# Autodesk Inventor assembly: V1Towers
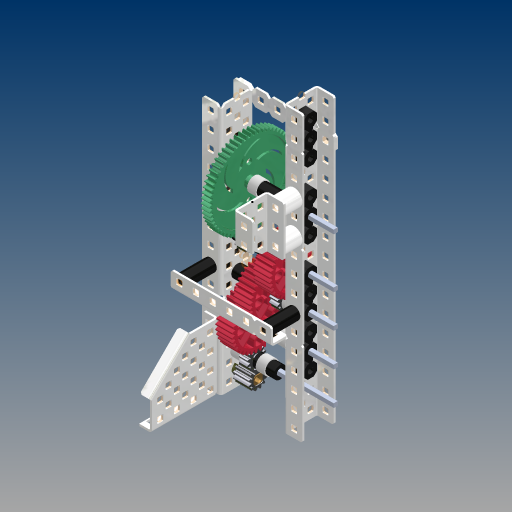
[picture p0: Inventor's stored thumbnail of the model, 512x512]
Saved by Autodesk Inventor 2023 (Build 270158000, 158)
## iProperties
Created: 2023-07-20
Part Number: V1Towers
Document SubType Name: Assembly
Designer: eddie
Author: eddie
## Documents named in this file (26)
- C:\Users\eddie\Documents\81208X-Over-Under-CAD\V1\V1Tower_Right.iam
- C:\Users\eddie\Documents\81208X-Over-Under-CAD\VEX-CAD-Inventor-1.4.0\Motion\Spacers\Spacer Nylon .375 OD\NSpacer .375 OD x .375.ipt
- C:\Users\eddie\Documents\81208X-Over-Under-CAD\VEX-CAD-Inventor-1.4.0\Motion\Spacers\Spacer Nylon .375 OD.ipt
- C:\Users\eddie\Documents\81208X-Over-Under-CAD\VEX-CAD-Inventor-1.4.0\Motion\Spacers\Spacer Nylon .375 OD\NSpacer .375 OD x .500.ipt
- C:\Users\eddie\Documents\81208X-Over-Under-CAD\VEX-CAD-Inventor-1.4.0\Motion\Spacers\Spacer Nylon .500 OD\NSpacer White .500 OD x .500.ipt
- C:\Users\eddie\Documents\81208X-Over-Under-CAD\VEX-CAD-Inventor-1.4.0\Motion\Spacers\Spacer Nylon .500 OD.ipt
- C:\Users\eddie\Documents\81208X-Over-Under-CAD\VEX-CAD-Inventor-1.4.0\Motion\Shaft LS\Shaft LS\Shaft LS 3.0.ipt
- C:\Users\eddie\Documents\81208X-Over-Under-CAD\VEX-CAD-Inventor-1.4.0\Motion\Shaft LS\Shaft LS.ipt
- C:\Users\eddie\Documents\81208X-Over-Under-CAD\VEX-CAD-Inventor-1.4.0\Motion\Spacers\Spacer Nylon .375 OD\NSpacer .375 OD x .125.ipt
- C:\Users\eddie\Documents\81208X-Over-Under-CAD\VEX-CAD-Inventor-1.4.0\Motion\Spacers\Spacer Nylon .375 OD\NSpacer .375 OD x .250.ipt
- C:\Users\eddie\Documents\81208X-Over-Under-CAD\VEX-CAD-Inventor-1.4.0\Motion\Spacers\Washer Steel\SWasher .375 OD x .031250.ipt
- C:\Users\eddie\Documents\81208X-Over-Under-CAD\VEX-CAD-Inventor-1.4.0\Motion\Spacers\Washer Steel.ipt
- C:\Users\eddie\Documents\81208X-Over-Under-CAD\Custom-parts\Angle Corner Gusset.ipt
- C:\Users\eddie\Documents\81208X-Over-Under-CAD\VEX-CAD-Inventor-1.4.0\Structure\C Channel\Aluminum 1x2x1\Alu C 1x2x1x15_MIR.ipt
- C:\Users\eddie\Documents\81208X-Over-Under-CAD\VEX-CAD-Inventor-1.4.0\Structure\C Channel\Aluminum 1x2x1\Alu C 1x2x1x17_MIR.ipt
- C:\Users\eddie\Documents\81208X-Over-Under-CAD\VEX-CAD-Inventor-1.4.0\Structure\Plate\Aluminum\Alu Plate 1x6_MIR.ipt
- C:\Users\eddie\Documents\81208X-Over-Under-CAD\VEX-CAD-Inventor-1.4.0\Structure\Angle\Aluminum\1x1\Alu Angle 1x1x6_MIR.ipt
- C:\Users\eddie\Documents\81208X-Over-Under-CAD\Custom-parts\3x2 channel triangular slice_MIR.ipt
- C:\Users\eddie\Documents\81208X-Over-Under-CAD\VEX-CAD-Inventor-1.4.0\Motion\Shaft LS\Bearing Flat_MIR1.ipt
- C:\Users\eddie\Documents\81208X-Over-Under-CAD\VEX-CAD-Inventor-1.4.0\Structure\Hardware\Nut Alu_MIR.ipt
- C:\Users\eddie\Documents\81208X-Over-Under-CAD\VEX-CAD-Inventor-1.4.0\Motion\Gears\HS Gear\HS 12T Gear, Circle_MIR.iam
- C:\Users\eddie\Documents\81208X-Over-Under-CAD\Custom-parts\Shaft Collar_MIR.ipt
- C:\Users\eddie\Documents\81208X-Over-Under-CAD\VEX-CAD-Inventor-1.4.0\Motion\Gears\LS 12T Gear Steel_MIR.ipt
- C:\Users\eddie\Documents\81208X-Over-Under-CAD\VEX-CAD-Inventor-1.4.0\Motion\Gears\HS Gear\HS 36T Gear, Square_MIR.iam
- C:\Users\eddie\Documents\81208X-Over-Under-CAD\VEX-CAD-Inventor-1.4.0\Motion\Gears\LS 60T Gear_MIR.ipt
- C:\Users\eddie\Documents\81208X-Over-Under-CAD\Custom-parts\Angle Corner Gusset_MIR.ipt
## Components (61 placed, 21 different names)
1. Angle Corner Gusset:1
2. Alu C 1x2x1x15_MIR:1 — Insert:61, Insert:62, Insert:70, Insert:71, Insert:72, Insert:73, Insert:78, Insert:85, Insert:91, Insert:98, Insert:105, Insert:112, Insert:118
3. Alu C 1x2x1x17_MIR:1 — Insert:60, Insert:64, Insert:67, Insert:68, Insert:74, Insert:75, Insert:76, Insert:77, Insert:90
4. Alu Plate 1x6_MIR:1 — Insert:60, Insert:61
5. NSpacer .375 OD x .375:23 — Insert:62, Insert:63
6. NSpacer .375 OD x .500:24 — Insert:63, Insert:66
7. NSpacer .375 OD x .375:25 — Insert:64, Insert:65
8. NSpacer .375 OD x .500:26 — Insert:65
9. Alu Angle 1x1x6_MIR:1 — Insert:66
10. NSpacer White .500 OD x .500:3 — Insert:67, Insert:69
11. NSpacer White .500 OD x .500:4 — Insert:68
12. 3x2 channel triangular slice_MIR:1 — Insert:69
13. Bearing Flat_MIR1:1 — Insert:70, Insert:82, Insert:83
14. Bearing Flat_MIR1:2 — Insert:71, Insert:81
15. Bearing Flat_MIR1:3 — Insert:72, Insert:84
16. Bearing Flat_MIR1:4 — Insert:73, Insert:80
17. Bearing Flat_MIR1:5 — Insert:74
18. Bearing Flat_MIR1:6 — Insert:75
19. Bearing Flat_MIR1:7 — Insert:76
20. Bearing Flat_MIR1:8 — Insert:77
21. Nut Alu_MIR:1 — Insert:78, Insert:79
22. HS 12T Gear, Circle_MIR:1 [sub-assembly] — Insert:79
23. Shaft LS 3.0:6 — Insert:80
24. Shaft LS 3.0:7 — Insert:81
25. Shaft LS 3.0:8 — Insert:82
26. Shaft LS 3.0:9 — Insert:83
27. Shaft LS 3.0:10 — Insert:84
28. Shaft Collar_MIR:1 — Insert:85, Insert:86
29. LS 12T Gear Steel_MIR:1 — Insert:86, Insert:87
30. NSpacer .375 OD x .125:27 — Insert:87, Insert:88
31. Shaft Collar_MIR:2 — Insert:88, Insert:89
32. NSpacer .375 OD x .250:28 — Insert:89
33. Bearing Flat_MIR1:9 — Insert:90
34. NSpacer .375 OD x .125:29 — Insert:91, Insert:92
35. HS 36T Gear, Square_MIR:1 [sub-assembly] — Insert:92, Insert:93
36. LS 12T Gear Steel_MIR:2 — Insert:93, Insert:94
37. NSpacer .375 OD x .375:30 — Insert:94, Insert:95
38. Shaft Collar_MIR:3 — Insert:95, Insert:96
39. NSpacer .375 OD x .125:31 — Insert:96, Insert:97
40. NSpacer .375 OD x .125:32 — Insert:97
41. NSpacer .375 OD x .500:33 — Insert:98, Insert:99
42. SWasher .375 OD x .031250:2 — Insert:99, Insert:100
43. NSpacer .375 OD x .125:34 — Insert:100, Insert:101
44. HS 36T Gear, Square_MIR:2 [sub-assembly] — Insert:101, Insert:102
45. LS 12T Gear Steel_MIR:3 — Insert:102, Insert:103
46. Shaft Collar_MIR:4 — Insert:103, Insert:104
47. NSpacer .375 OD x .125:35 — Insert:104
48. NSpacer .375 OD x .125:36 — Insert:105, Insert:106
49. LS 60T Gear_MIR:1 — Insert:106, Insert:107
50. Shaft Collar_MIR:5 — Insert:107, Insert:108
51. NSpacer .375 OD x .375:37 — Insert:108, Insert:110
52. NSpacer .375 OD x .375:38 — Insert:109, Insert:111
53. NSpacer .375 OD x .250:39 — Insert:109, Insert:110
54. NSpacer .375 OD x .125:40 — Insert:111
55. NSpacer .375 OD x .250:41 — Insert:114, Insert:116
56. NSpacer .375 OD x .125:42 — Insert:112, Insert:113
57. LS 12T Gear Steel_MIR:4 — Insert:113, Insert:115
58. NSpacer .375 OD x .500:43 — Insert:114, Insert:115
59. HS 36T Gear, Square_MIR:3 [sub-assembly] — Insert:116, Insert:117
60. NSpacer .375 OD x .125:44 — Insert:117
61. Angle Corner Gusset_MIR:1 — Insert:118
## Relationships (59: Insert 59)
- Insert:60: Alu C 1x2x1x17_MIR:1 ↔ Alu Plate 1x6_MIR:1
- Insert:61: Alu C 1x2x1x15_MIR:1 ↔ Alu Plate 1x6_MIR:1
- Insert:62: Alu C 1x2x1x15_MIR:1 ↔ NSpacer .375 OD x .375:23
- Insert:63: NSpacer .375 OD x .375:23 ↔ NSpacer .375 OD x .500:24
- Insert:64: Alu C 1x2x1x17_MIR:1 ↔ NSpacer .375 OD x .375:25
- Insert:65: NSpacer .375 OD x .375:25 ↔ NSpacer .375 OD x .500:26
- Insert:66: NSpacer .375 OD x .500:24 ↔ Alu Angle 1x1x6_MIR:1
- Insert:67: Alu C 1x2x1x17_MIR:1 ↔ NSpacer White .500 OD x .500:3
- Insert:68: Alu C 1x2x1x17_MIR:1 ↔ NSpacer White .500 OD x .500:4
- Insert:69: NSpacer White .500 OD x .500:3 ↔ 3x2 channel triangular slice_MIR:1
- Insert:70: Alu C 1x2x1x15_MIR:1 ↔ Bearing Flat_MIR1:1
- Insert:71: Alu C 1x2x1x15_MIR:1 ↔ Bearing Flat_MIR1:2
- Insert:72: Alu C 1x2x1x15_MIR:1 ↔ Bearing Flat_MIR1:3
- Insert:73: Alu C 1x2x1x15_MIR:1 ↔ Bearing Flat_MIR1:4
- Insert:74: Alu C 1x2x1x17_MIR:1 ↔ Bearing Flat_MIR1:5
- Insert:75: Alu C 1x2x1x17_MIR:1 ↔ Bearing Flat_MIR1:6
- Insert:76: Alu C 1x2x1x17_MIR:1 ↔ Bearing Flat_MIR1:7
- Insert:77: Alu C 1x2x1x17_MIR:1 ↔ Bearing Flat_MIR1:8
- Insert:78: Alu C 1x2x1x15_MIR:1 ↔ Nut Alu_MIR:1
- Insert:79: Nut Alu_MIR:1 ↔ HS 12T Gear, Circle_MIR:1
- Insert:80: Bearing Flat_MIR1:4 ↔ Shaft LS 3.0:6
- Insert:81: Bearing Flat_MIR1:2 ↔ Shaft LS 3.0:7
- Insert:82: Bearing Flat_MIR1:1 ↔ Shaft LS 3.0:8
- Insert:83: Bearing Flat_MIR1:1 ↔ Shaft LS 3.0:9
- Insert:84: Bearing Flat_MIR1:3 ↔ Shaft LS 3.0:10
- Insert:85: Alu C 1x2x1x15_MIR:1 ↔ Shaft Collar_MIR:1
- Insert:86: Shaft Collar_MIR:1 ↔ LS 12T Gear Steel_MIR:1
- Insert:87: LS 12T Gear Steel_MIR:1 ↔ NSpacer .375 OD x .125:27
- Insert:88: NSpacer .375 OD x .125:27 ↔ Shaft Collar_MIR:2
- Insert:89: Shaft Collar_MIR:2 ↔ NSpacer .375 OD x .250:28
- Insert:90: Alu C 1x2x1x17_MIR:1 ↔ Bearing Flat_MIR1:9
- Insert:91: Alu C 1x2x1x15_MIR:1 ↔ NSpacer .375 OD x .125:29
- Insert:92: NSpacer .375 OD x .125:29 ↔ HS 36T Gear, Square_MIR:1
- Insert:93: HS 36T Gear, Square_MIR:1 ↔ LS 12T Gear Steel_MIR:2
- Insert:94: LS 12T Gear Steel_MIR:2 ↔ NSpacer .375 OD x .375:30
- Insert:95: NSpacer .375 OD x .375:30 ↔ Shaft Collar_MIR:3
- Insert:96: Shaft Collar_MIR:3 ↔ NSpacer .375 OD x .125:31
- Insert:97: NSpacer .375 OD x .125:31 ↔ NSpacer .375 OD x .125:32
- Insert:98: Alu C 1x2x1x15_MIR:1 ↔ NSpacer .375 OD x .500:33
- Insert:99: NSpacer .375 OD x .500:33 ↔ SWasher .375 OD x .031250:2
- Insert:100: SWasher .375 OD x .031250:2 ↔ NSpacer .375 OD x .125:34
- Insert:101: NSpacer .375 OD x .125:34 ↔ HS 36T Gear, Square_MIR:2
- Insert:102: HS 36T Gear, Square_MIR:2 ↔ LS 12T Gear Steel_MIR:3
- Insert:103: LS 12T Gear Steel_MIR:3 ↔ Shaft Collar_MIR:4
- Insert:104: Shaft Collar_MIR:4 ↔ NSpacer .375 OD x .125:35
- Insert:105: Alu C 1x2x1x15_MIR:1 ↔ NSpacer .375 OD x .125:36
- Insert:106: NSpacer .375 OD x .125:36 ↔ LS 60T Gear_MIR:1
- Insert:107: LS 60T Gear_MIR:1 ↔ Shaft Collar_MIR:5
- Insert:108: Shaft Collar_MIR:5 ↔ NSpacer .375 OD x .375:37
- Insert:109: NSpacer .375 OD x .375:38 ↔ NSpacer .375 OD x .250:39
- Insert:110: NSpacer .375 OD x .375:37 ↔ NSpacer .375 OD x .250:39
- Insert:111: NSpacer .375 OD x .375:38 ↔ NSpacer .375 OD x .125:40
- Insert:112: Alu C 1x2x1x15_MIR:1 ↔ NSpacer .375 OD x .125:42
- Insert:113: NSpacer .375 OD x .125:42 ↔ LS 12T Gear Steel_MIR:4
- Insert:114: NSpacer .375 OD x .250:41 ↔ NSpacer .375 OD x .500:43
- Insert:115: LS 12T Gear Steel_MIR:4 ↔ NSpacer .375 OD x .500:43
- Insert:116: NSpacer .375 OD x .250:41 ↔ HS 36T Gear, Square_MIR:3
- Insert:117: HS 36T Gear, Square_MIR:3 ↔ NSpacer .375 OD x .125:44
- Insert:118: Alu C 1x2x1x15_MIR:1 ↔ Angle Corner Gusset_MIR:1
